# Autodesk Inventor assembly: UpperArm
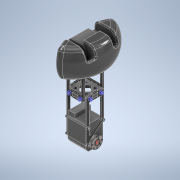
[picture p0: Inventor's stored thumbnail of the model, 180x180]
Saved by Autodesk Inventor 2022 (Build 260153000, 153)
## iProperties
Created: 2023-09-11
Part Number: UpperArm
Document SubType Name: Assembly
Designer: Masato Kubotera
Author: Masato Kubotera
## Documents named in this file (3)
- C:\Users\MasatoKubotera\Documents\Inventor\SUSTAINA-OP\UpperBody\Arm\UpperArm.iam
- C:\Users\MasatoKubotera\Documents\Inventor\SUSTAINA-OP\UpperBody\Arm\SideBumper.ipt
- C:\Users\MasatoKubotera\Documents\Inventor\SUSTAINA-OP\UpperBody\Arm\UpperArm_without_bumper.iam
## Components (2 placed, 2 different names)
1. SideBumper:1 — フラッシュ:4, フラッシュ:5, フラッシュ:6
2. UpperArm_without_bumper:1 [sub-assembly] — フラッシュ:1, フラッシュ:2, フラッシュ:4, フラッシュ:5, フラッシュ:6, メイト:1
## Relationships (6: Flush 5, Mate 1)
- フラッシュ:1 [Flush]: UpperArm_without_bumper:1
- フラッシュ:2 [Flush]: UpperArm_without_bumper:1
- フラッシュ:4 [Flush]: SideBumper:1 ↔ UpperArm_without_bumper:1
- フラッシュ:5 [Flush]: SideBumper:1 ↔ UpperArm_without_bumper:1
- フラッシュ:6 [Flush]: SideBumper:1 ↔ UpperArm_without_bumper:1
- メイト:1 [Mate]: UpperArm_without_bumper:1
